# Autodesk Inventor assembly: Gimbal Assembly
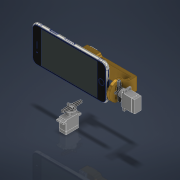
[picture p0: Inventor's stored thumbnail of the model, 180x180]
Saved by Autodesk Inventor 2022 (Build 260153000, 153)
## iProperties
Created: 2021-07-30
Part Number: Gimbal Assembly
Document SubType Name: Assembly
Designer: sidsa
Author: sidsa
## Documents named in this file (4)
- D:\My Documents\gitHUB Rocketry\mlh-selfie-hacks\CAD Models\Gimbal Assembly.iam
- D:\My Documents\gitHUB Rocketry\mlh-selfie-hacks\CAD Models\Mg90 Servo\MG90servo_assembly.ipt
- D:\My Documents\gitHUB Rocketry\mlh-selfie-hacks\CAD Models\iPhone\iphone 6.ipt
- D:\My Documents\gitHUB Rocketry\mlh-selfie-hacks\CAD Models\Roll Pitch Axis Support.ipt
## Components (5 placed, 3 different names)
1. MG90servo_assembly:3
2. iphone 6:1 — Mate:1
3. MG90servo_assembly:4 — Mate:1, Mate:2, Flush:1, Mate:3
4. MG90servo_assembly:5 — Mate:4, Mate:5
5. Roll Pitch Axis Support:1 — Mate:2, Flush:1, Mate:3, Mate:4, Mate:5
## Relationships (6: Mate 5, Flush 1)
- Mate:1: iphone 6:1 ↔ MG90servo_assembly:4
- Mate:2: MG90servo_assembly:4 ↔ Roll Pitch Axis Support:1
- Flush:1: MG90servo_assembly:4 ↔ Roll Pitch Axis Support:1
- Mate:3: MG90servo_assembly:4 ↔ Roll Pitch Axis Support:1
- Mate:4: MG90servo_assembly:5 ↔ Roll Pitch Axis Support:1
- Mate:5: MG90servo_assembly:5 ↔ Roll Pitch Axis Support:1
